# Autodesk Inventor assembly: nsyspf10100
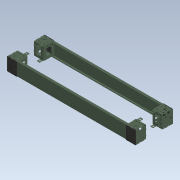
[picture p0: Inventor's stored thumbnail of the model, 180x180]
Saved by Autodesk Inventor 2021 (Build 250183000, 183)
## iProperties
Created: 2018-05-29
Part Number: nsyspf10100
Checked By: TraceParts S.A.
Catalog Web Link: www.traceparts.com
Document SubType Name: Assembly
Designer: TraceParts
Company: TraceParts S.A.
REFERENCE: NSYSPF10100
SUPPLIER: Schneider Electric
DESIGN: Zócalo frontal para Spacial SF-SM, 1000x100
OMNICLASS23: 23.35.33.15
TraceParts.PartVersion: 1.3.5
TraceParts.PartStatus: Published
TraceParts.PartNumber: 10-20052009-115852
TraceParts.PartLanguage: es
TraceParts.InstanceId: 10-20052009-1158525Z4UCOFAJ4JO7OEJHY0I1IE0F
TraceParts.PartTitle: Zócalo frontal para Spacial SF-SM
TRACEPARTS: TRACEPARTS
TraceParts.ClassPath: SCHNEIDER_ELECTRIC_DISTRI:/SCHNEIDER_DISTRI/F_SCHNEIDER_ELECTRIC_ENVEL/SCHNEIDER_ELECTRIC_ENVEL.110/SCHNEIDER_ELECTRIC_ENVEL.110.010/SCHNEIDER_ELECTRIC_ENVEL.110.010.100/SCHNEIDER_ELECTRIC_ENVEL.110.010.100.020/10-20052009-115852
Author: TraceParts
## Documents named in this file (11)
- C:\Users\andre\Documents\GitHub\Dis.-Mecatronico-E6\inventor proyecto\Tablero\Armario\nsyspf10100.iam
- C:\Users\andre\Documents\GitHub\Dis.-Mecatronico-E6\inventor proyecto\Tablero\Armario\nsyspf10100_01.ipt
- C:\Users\andre\Documents\GitHub\Dis.-Mecatronico-E6\inventor proyecto\Tablero\Armario\nsyspf10100_02.ipt
- C:\Users\andre\Documents\GitHub\Dis.-Mecatronico-E6\inventor proyecto\Tablero\Armario\nsyspf10100_03.ipt
- C:\Users\andre\Documents\GitHub\Dis.-Mecatronico-E6\inventor proyecto\Tablero\Armario\nsyspf10100_04.ipt
- C:\Users\andre\Documents\GitHub\Dis.-Mecatronico-E6\inventor proyecto\Tablero\Armario\nsyspf10100_05.ipt
- C:\Users\andre\Documents\GitHub\Dis.-Mecatronico-E6\inventor proyecto\Tablero\Armario\nsyspf10100_06.ipt
- C:\Users\andre\Documents\GitHub\Dis.-Mecatronico-E6\inventor proyecto\Tablero\Armario\nsyspf10100_07.ipt
- C:\Users\andre\Documents\GitHub\Dis.-Mecatronico-E6\inventor proyecto\Tablero\Armario\nsyspf10100_08.ipt
- C:\Users\andre\Documents\GitHub\Dis.-Mecatronico-E6\inventor proyecto\Tablero\Armario\nsyspf10100_09.ipt
- C:\Users\andre\Documents\GitHub\Dis.-Mecatronico-E6\inventor proyecto\Tablero\Armario\nsyspf10100_10.ipt
## Components (10 placed, 10 different names)
1. nsyspf10100_01:1 — Mate:1, Rigid:1, Rigid:2
2. nsyspf10100_02:1 — Flush:1, Rigid:2, Mate:3, Flush:6, Flush:7
3. nsyspf10100_03:1 — Rigid:1, Mate:2, Flush:2, Flush:3, Flush:4, Flush:5
4. nsyspf10100_04:1 — Mate:3, Flush:6, Flush:7
5. nsyspf10100_05:1 — Mate:2, Flush:2, Flush:3
6. nsyspf10100_06:1 — Mate:1
7. nsyspf10100_07:1 — Flush:4, Flush:5
8. nsyspf10100_08:1 — Flush:1
9. nsyspf10100_09:1
10. nsyspf10100_10:1
## Relationships (12: Flush 7, Mate 3, WeldJoint 2)
- Mate:1 (500 mm): nsyspf10100_01:1 ↔ nsyspf10100_06:1
- Flush:1: nsyspf10100_02:1 ↔ nsyspf10100_08:1
- Rigid:1 [WeldJoint]: nsyspf10100_01:1 ↔ nsyspf10100_03:1
- Mate:2: nsyspf10100_03:1 ↔ nsyspf10100_05:1
- Flush:2: nsyspf10100_03:1 ↔ nsyspf10100_05:1
- Flush:3: nsyspf10100_03:1 ↔ nsyspf10100_05:1
- Flush:4: nsyspf10100_03:1 ↔ nsyspf10100_07:1
- Flush:5: nsyspf10100_03:1 ↔ nsyspf10100_07:1
- Rigid:2 [WeldJoint]: nsyspf10100_01:1 ↔ nsyspf10100_02:1
- Mate:3: nsyspf10100_02:1 ↔ nsyspf10100_04:1
- Flush:6: nsyspf10100_02:1 ↔ nsyspf10100_04:1
- Flush:7: nsyspf10100_02:1 ↔ nsyspf10100_04:1
